# Autodesk Inventor assembly: DriveSubassembly
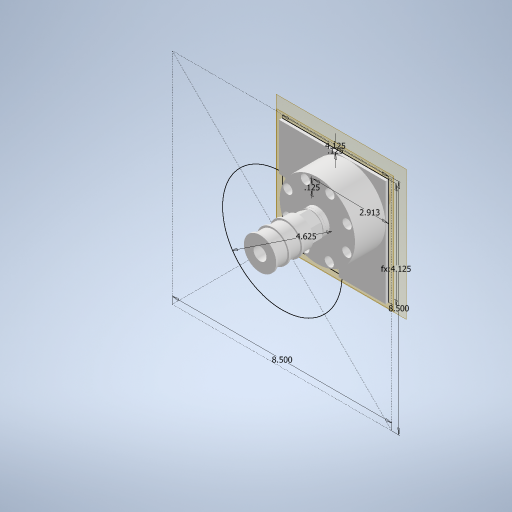
[picture p0: Inventor's stored thumbnail of the model, 512x512]
Saved by Autodesk Inventor 2024 (Build 280153000, 153)
## iProperties
Created: 2024-12-18
Part Number: DriveSubassembly
Document SubType Name: Assembly
Designer: Tommy Rohmann
Author: Tommy Rohmann
## Documents named in this file (7)
- C:\Users\Tommy Rohmann\OneDrive\Projects\Microgravity-Press-Washing-Machine\System Design and Documentation\Inventor Design Project\DriveSubassembly.iam
- C:\Users\Tommy Rohmann\OneDrive\Projects\Microgravity-Press-Washing-Machine\System Design and Documentation\Inventor Design Project\LoadCellBase.ipt
- C:\Users\Tommy Rohmann\OneDrive\Projects\Microgravity-Press-Washing-Machine\System Design and Documentation\Inventor Design Project\BearingBaseA.ipt
- C:\Users\Tommy Rohmann\OneDrive\Projects\Microgravity-Press-Washing-Machine\System Design and Documentation\Inventor Design Project\LoadCell.ipt
- C:\Users\Tommy Rohmann\OneDrive\Projects\Microgravity-Press-Washing-Machine\System Design and Documentation\Inventor Design Project\ACMEHexNut.ipt
- C:\Users\Tommy Rohmann\OneDrive\Projects\Microgravity-Press-Washing-Machine\System Design and Documentation\Inventor Design Project\ThrustBearing.ipt
- C:\Users\Tommy Rohmann\OneDrive\Projects\Microgravity-Press-Washing-Machine\System Design and Documentation\Inventor Design Project\FlangedJournalBearing.ipt
## Components (11 placed, 6 different names)
1. LoadCellBase:1 — Mate:1, Mate:2
2. BearingBaseA:1 — Flush:1, Flush:2
3. LoadCell:1 — Mate:1, Mate:2, Mate:3, Mate:4, Mate:5, Mate:6, Mate:7, Mate:8
4. ACMEHexNut:1 — Mate:4, Mate:9, Mate:11, Mate:13, Mate:14
5. ACMEHexNut:2 — Mate:3, Mate:10, Mate:12
6. ThrustBearing:1 — Mate:6, Mate:7, Mate:10
7. ThrustBearing:2 — Mate:5, Mate:8, Mate:9
8. FlangedJournalBearing:1 — Mate:11, Mate:14, Mate:15, Mate:17
9. FlangedJournalBearing:2 — Mate:12, Mate:13
10. FlangedJournalBearing:3 — Mate:15, Mate:16, Mate:17, Mate:18
11. FlangedJournalBearing:4 — Mate:16, Mate:18
## Relationships (20: Mate 18, Flush 2)
- Flush:1: BearingBaseA:1
- Flush:2: BearingBaseA:1
- Mate:1: LoadCellBase:1 ↔ LoadCell:1
- Mate:2: LoadCellBase:1 ↔ LoadCell:1
- Mate:3: LoadCell:1 ↔ ACMEHexNut:2
- Mate:4: LoadCell:1 ↔ ACMEHexNut:1
- Mate:5: LoadCell:1 ↔ ThrustBearing:2
- Mate:6: LoadCell:1 ↔ ThrustBearing:1
- Mate:7: LoadCell:1 ↔ ThrustBearing:1
- Mate:8: LoadCell:1 ↔ ThrustBearing:2
- Mate:9: ACMEHexNut:1 ↔ ThrustBearing:2
- Mate:10: ACMEHexNut:2 ↔ ThrustBearing:1
- Mate:11: ACMEHexNut:1 ↔ FlangedJournalBearing:1
- Mate:12: ACMEHexNut:2 ↔ FlangedJournalBearing:2
- Mate:13: ACMEHexNut:1 ↔ FlangedJournalBearing:2
- Mate:14: ACMEHexNut:1 ↔ FlangedJournalBearing:1
- Mate:15: FlangedJournalBearing:1 ↔ FlangedJournalBearing:3
- Mate:16: FlangedJournalBearing:3 ↔ FlangedJournalBearing:4
- Mate:17: FlangedJournalBearing:1 ↔ FlangedJournalBearing:3
- Mate:18: FlangedJournalBearing:3 ↔ FlangedJournalBearing:4
## Named parameters: FootprintSizeLimit = 215.9 mm
